# Autodesk Inventor assembly: ASY Мешалка
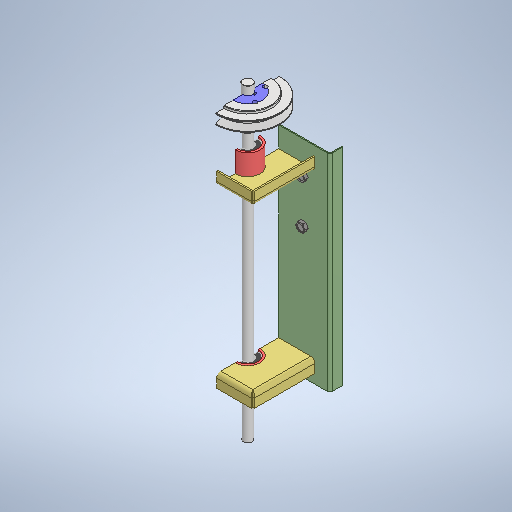
[picture p0: Inventor's stored thumbnail of the model, 512x512]
Saved by Autodesk Inventor 2025 (Build 290162010, 162A)
## iProperties
Created: 2024-04-09
Part Number: ASY Мешалка
Document SubType Name: Assembly
Designer: pokla
Stock Number: ASY Мешалка
Author: pokla
## Documents named in this file (12)
- C:\Users\pokla\Documents\Inventor\Gusev_Meshalka\ASY Мешалка\ASY Мешалка.iam
- C:\Users\pokla\Documents\Inventor\Gusev_Meshalka\ASY Мешалка\SKF B7203 BE.ipt
- C:\Users\pokla\Documents\Inventor\Gusev_Meshalka\ASY Мешалка\CSN 02 9401 - G 17x40x7 - NBR.ipt
- C:\Users\pokla\Documents\Inventor\Gusev_Meshalka\ASY Мешалка\Шкив 119 мм.ipt
- Шкив 119 мм.ipt
- C:\Users\pokla\Documents\Inventor\Gusev_Meshalka\ASY Мешалка\Втулка для шкива.ipt
- C:\Users\pokla\Documents\Inventor\Gusev_Meshalka\ASY Мешалка\ANSI B 27.7M - 3AMI-17.ipt
- C:\Users\pokla\Documents\Inventor\Gusev_Meshalka\ASY Мешалка\ANSI B 27.7M - 3BMI-40.ipt
- C:\Users\pokla\Documents\Inventor\Gusev_Meshalka\ASY Мешалка\Корпус.iam
- C:\Users\pokla\Documents\Inventor\Gusev_Meshalka\ASY Мешалка\Седло для подшипника.ipt
- C:\Users\pokla\Documents\Inventor\Gusev_Meshalka\ASY Мешалка\Shaft1.ipt
- C:\Users\pokla\Documents\Inventor\Gusev_Meshalka\ASY Мешалка\Крепление корпуса.ipt
## Components (19 placed, 15 different names)
1. SKF B7203 BE.ipt:1 — Rigid:22, Mate:7
2. CSN 02 9401 - G 17x40x7 - NBR.ipt:2 — Cylindrical:1, Mate:9
3. Шкив 119 мм.ipt:1 — Rigid:18
4. Втулка для шкива.ipt:1 — Rigid:18, Rigid:19
5. ANSI B 27.7M - 3AMI-17.ipt:1 — Rigid:15, Mate:7
6. ANSI B 27.7M - 3BMI-40.ipt:2 — Rigid:24, Mate:10
7. Крепление корпуса.ipt:1 — Flush:5, Mate:3, Flush:6, Rigid:20
8. Корпус.iam:1 [sub-assembly] — Flush:1, Flush:2, Flush:3, Flush:4, Mate:1, Flush:5, Mate:3
9. Седло для подшипника.ipt:1 — Rigid:20, Mate:4, Rigid:22, Rigid:24, Rigid:25
10. Shaft:1 — Rigid:15, Rigid:19, Mate:4, Mate:6, Cylindrical:1, Cylindrical:2, Cylindrical:3
11. Крепление корпуса:2 — Flush:4, Mate:1, Mate:2, Rigid:21
12. Седло для подшипника:2 — Rigid:21, Rigid:23, Rigid:26, Rigid:27
13. CSN 02 9401 G G 17x40x7 - NBR:3 — Mate:6, Mate:8
14. SKF B- Angular contact SKF B7203 BE:4 — Rigid:23
15. CSN 02 9401 G G 17x40x7 - NBR:4 — Cylindrical:2, Mate:10
16. ANSI B 27.7M 3BMI-40:3 — Rigid:25, Mate:9
17. ANSI B 27.7M 3BMI-40:4 — Rigid:26, Mate:11
18. ANSI B 27.7M 3BMI-40:5 — Rigid:27, Mate:8
19. CSN 02 9401 G G 17x40x7 - NBR:5 — Cylindrical:3, Mate:11
## Relationships (30: WeldJoint 11, Mate 10, Flush 6, CylindricalJoint 3)
- Flush:1: Корпус.iam:1
- Flush:2: Корпус.iam:1
- Flush:3: Корпус.iam:1
- Rigid:15 [WeldJoint]: ANSI B 27.7M - 3AMI-17.ipt:1 ↔ Shaft:1
- Rigid:18 [WeldJoint]: Шкив 119 мм.ipt:1 ↔ Втулка для шкива.ipt:1
- Rigid:19 [WeldJoint] (-16.3 mm): Втулка для шкива.ipt:1 ↔ Shaft:1
- Flush:4 (18 mm): Корпус.iam:1 ↔ Крепление корпуса:2
- Mate:1: Корпус.iam:1 ↔ Крепление корпуса:2
- Mate:2: Крепление корпуса:2
- Flush:5 (18 mm): Крепление корпуса.ipt:1 ↔ Корпус.iam:1
- Mate:3: Крепление корпуса.ipt:1 ↔ Корпус.iam:1
- Flush:6: Крепление корпуса.ipt:1
- Rigid:20 [WeldJoint]: Крепление корпуса.ipt:1 ↔ Седло для подшипника.ipt:1
- Rigid:21 [WeldJoint]: Крепление корпуса:2 ↔ Седло для подшипника:2
- Mate:4: Седло для подшипника.ipt:1 ↔ Shaft:1
- Mate:6: Shaft:1 ↔ CSN 02 9401 G G 17x40x7 - NBR:3
- Rigid:22 [WeldJoint]: SKF B7203 BE.ipt:1 ↔ Седло для подшипника.ipt:1
- Rigid:23 [WeldJoint]: Седло для подшипника:2 ↔ SKF B- Angular contact SKF B7203 BE:4
- Mate:7: SKF B7203 BE.ipt:1 ↔ ANSI B 27.7M - 3AMI-17.ipt:1
- Rigid:24 [WeldJoint]: ANSI B 27.7M - 3BMI-40.ipt:2 ↔ Седло для подшипника.ipt:1
- Rigid:25 [WeldJoint]: Седло для подшипника.ipt:1 ↔ ANSI B 27.7M 3BMI-40:3
- Rigid:26 [WeldJoint]: Седло для подшипника:2 ↔ ANSI B 27.7M 3BMI-40:4
- Rigid:27 [WeldJoint]: Седло для подшипника:2 ↔ ANSI B 27.7M 3BMI-40:5
- Cylindrical:1: CSN 02 9401 - G 17x40x7 - NBR.ipt:2 ↔ Shaft:1
- Mate:8: CSN 02 9401 G G 17x40x7 - NBR:3 ↔ ANSI B 27.7M 3BMI-40:5
- Mate:9: CSN 02 9401 - G 17x40x7 - NBR.ipt:2 ↔ ANSI B 27.7M 3BMI-40:3
- Cylindrical:2: Shaft:1 ↔ CSN 02 9401 G G 17x40x7 - NBR:4
- Mate:10: ANSI B 27.7M - 3BMI-40.ipt:2 ↔ CSN 02 9401 G G 17x40x7 - NBR:4
- Cylindrical:3: Shaft:1 ↔ CSN 02 9401 G G 17x40x7 - NBR:5
- Mate:11: ANSI B 27.7M 3BMI-40:4 ↔ CSN 02 9401 G G 17x40x7 - NBR:5
